# Autodesk Inventor assembly: Montagem_01
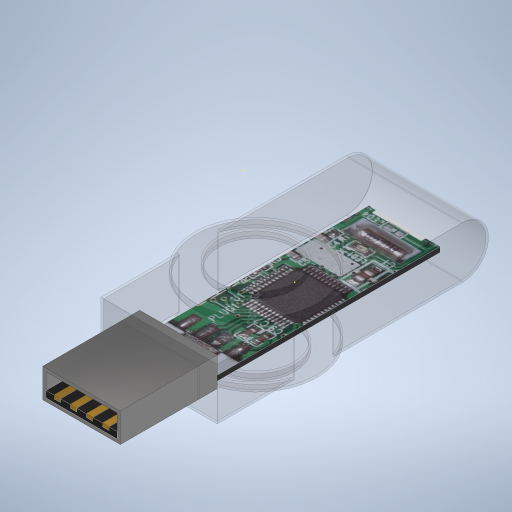
[picture p0: Inventor's stored thumbnail of the model, 512x512]
Saved by Autodesk Inventor 2024.2 (Build 282272000, 272)
## iProperties
Created: 2024-04-22
Part Number: Montagem_01
Document SubType Name: Assembly
Designer: 082220022
Author: 082220022
## Documents named in this file (5)
- Z:\2024 - 4S\Nilson\Projetos Inventor\Montagem_01.iam
- Z:\2024 - 4S\Nilson\Projetos Inventor\capa.ipt
- Z:\2024 - 4S\Nilson\Projetos Inventor\Pen2.ipt
- Z:\2024 - 4S\Nilson\Projetos Inventor\pen3_barra.ipt
- Z:\2024 - 4S\Nilson\Projetos Inventor\Pendrive.ipt
## Components (7 placed, 4 different names)
1. capa:1 — Mate:4, Flush:4, Mate:5, Flush:5, Mate:6, Mate:7
2. Pen2:1 — Mate:2, Flush:3, Mate:3, Mate:4, Flush:4, Mate:5
3. Pendrive:1 — Mate:1, Flush:1, Flush:2, Flush:5, Mate:6, Mate:7
4. pen3_barra:1 — Mate:2, Flush:3, Mate:3
5. pen3_barra:2
6. pen3_barra:3
7. pen3_barra:4
## Component patterns: (4 elements, first: pen3_barra:1)
## Relationships (12: Mate 7, Flush 5)
- Mate:1: Pendrive:1
- Flush:1: Pendrive:1
- Flush:2: Pendrive:1
- Mate:2: Pen2:1 ↔ pen3_barra:1
- Flush:3: Pen2:1 ↔ pen3_barra:1
- Mate:3: Pen2:1 ↔ pen3_barra:1
- Mate:4: capa:1 ↔ Pen2:1
- Flush:4: capa:1 ↔ Pen2:1
- Mate:5: capa:1 ↔ Pen2:1
- Flush:5 (-12 mm): capa:1 ↔ Pendrive:1
- Mate:6: capa:1 ↔ Pendrive:1
- Mate:7: capa:1 ↔ Pendrive:1
